# Autodesk Inventor assembly: beercart assembly - mekatronik
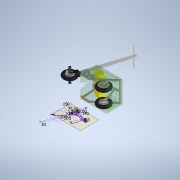
[picture p0: Inventor's stored thumbnail of the model, 180x180]
Saved by Autodesk Inventor 2022.2 (Build 262287000, 287)
## iProperties
_SolveAssemblyDoc: Frame Generator Solve Assembly
_Version: 15.0.0
Created: 2022-03-11
Part Number: beercart assembly - mekatronik
Document SubType Name: Assembly
Designer: foriw
Mass: 18232.1 g
Surface Area: 22436.3 cm^2
Volume: 9557.89 cm^3
Density: 1.90755 g/cm^3
Author: foriw
## Documents named in this file (15)
- H:\inventor ting\Mekatronik beercart git\Beercart CAD\Workspaces\Workspace\beercart assembly - mekatronik.iam
- H:\inventor ting\Mekatronik beercart git\Beercart CAD\Workspaces\Workspace\beercart- framwork - baseSketch.ipt
- H:\inventor ting\Mekatronik beercart git\Beercart CAD\Workspaces\Workspace\beercart assembly - mekatronik\Frame\Frame 1647030135921.iam
- H:\inventor ting\Mekatronik beercart git\Beercart CAD\Workspaces\Workspace\beer crate.ipt
- H:\inventor ting\Mekatronik beercart git\Beercart CAD\Workspaces\Workspace\Mekatronik-beerCart\frontwheel frame.ipt
- H:\inventor ting\Mekatronik beercart git\Beercart CAD\Workspaces\Workspace\motor at24v_MIR.ipt
- H:\inventor ting\Mekatronik beercart git\Beercart CAD\Workspaces\Workspace\FreeBackWheel.ipt
- H:\inventor ting\Mekatronik beercart git\Beercart CAD\Libraries\Content Center Files\en-US\ANSI B18.2.4.4M\ANSI B18.2.4.4M - M8 x 1,25.ipt
- H:\inventor ting\Mekatronik beercart git\Beercart CAD\Libraries\Content Center Files\en-US\DIN 6923\DIN 6923 - M8 x 1.25.ipt
- H:\inventor ting\Mekatronik beercart git\Beercart CAD\Workspaces\Workspace\Battery box.iam
- H:\inventor ting\Mekatronik beercart git\Beercart CAD\Workspaces\Workspace\beercart assembly - mekatronik\AIP\FEA\dxkkndp9c.fins
- H:\inventor ting\Mekatronik beercart git\Beercart CAD\Workspaces\Workspace\beercart assembly - mekatronik\AIP\FEA\dxkkndp9c.fsat
- H:\inventor ting\Mekatronik beercart git\Beercart CAD\Workspaces\Workspace\beercart assembly - mekatronik\AIP\FEA\dxkkndp9c.ftes
- H:\inventor ting\Mekatronik beercart git\Beercart CAD\Workspaces\Workspace\beercart assembly - mekatronik\AIP\FEA\dxkkndpa8.fwiz
- H:\inventor ting\Mekatronik beercart git\Beercart CAD\Workspaces\Workspace\beercart assembly - mekatronik\AIP\FEA\dxkkndpfk.fmsh
## Components (10 placed, 9 different names)
1. beercart- framwork - baseSketch:1
2. Frame 1647030135921:1 [sub-assembly] — Flush:3, Insert:2, Insert:3, Mate:3, Insert:5, Angle:1, Insert:6, Insert:7, Insert:8, Angle:2, Angle:9, Angle:3, Insert:9, Mate:4, Flush:6
3. frontwheel frame:1
4. beer crate:1 — Flush:2, Flush:3
5. motor at24v_MIR:1 — Insert:2, Insert:3, Mate:1, Insert:5, Angle:1, Tangent:1
6. FreeBackWheel:1 — Mate:1, Mate:3
7. Metric Hex Flange Nuts - Metric M8 x 1,25:1 — Insert:8
8. DIN 6923 M8:1 — Insert:6
9. DIN 6923 M8:2 — Insert:7, Insert:9
10. Battery box:1 [sub-assembly] — Angle:9, Angle:3, Mate:4, Flush:6
## Relationships (21: Insert 8, Flush 5, Angle 4, Mate 3, Tangent 1)
- Flush:2: beer crate:1
- Flush:3: Frame 1647030135921:1 ↔ beer crate:1
- [Insert]: Frame 1647030135921:1 ↔ motor at24v_MIR:1
- Insert:2: Frame 1647030135921:1 ↔ motor at24v_MIR:1
- Insert:3: Frame 1647030135921:1 ↔ motor at24v_MIR:1
- Mate:1: motor at24v_MIR:1 ↔ FreeBackWheel:1
- Mate:3 (0.5 mm): Frame 1647030135921:1 ↔ FreeBackWheel:1
- Insert:5: Frame 1647030135921:1 ↔ motor at24v_MIR:1
- Angle:1 (0 deg): Frame 1647030135921:1 ↔ motor at24v_MIR:1
- Insert:6: Frame 1647030135921:1 ↔ DIN 6923 M8:1
- [Flush]: frontwheel frame:1
- Insert:7: Frame 1647030135921:1 ↔ DIN 6923 M8:2
- Insert:8: Frame 1647030135921:1 ↔ Metric Hex Flange Nuts - Metric M8 x 1,25:1
- Angle:2 (0 deg): Frame 1647030135921:1
- Tangent:1: motor at24v_MIR:1
- Angle:9 (0 deg): Frame 1647030135921:1 ↔ Battery box:1
- Angle:3 (90 deg): Frame 1647030135921:1 ↔ Battery box:1
- Insert:9: Frame 1647030135921:1 ↔ DIN 6923 M8:2
- [Flush]: Frame 1647030135921:1
- Mate:4: Frame 1647030135921:1 ↔ Battery box:1
- Flush:6: Frame 1647030135921:1 ↔ Battery box:1
## Named parameters: sa_0 = 0, sa_1 = -148100, sa_2 = 0
note: some values were not read from the file. Shown as the stored number, unit unknown: "sa_0", "sa_1", "sa_2".
